# Autodesk Inventor assembly: 飛び出す奴
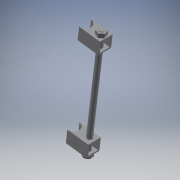
[picture p0: Inventor's stored thumbnail of the model, 180x180]
Saved by Autodesk Inventor 2018 (Build 220112000, 112)
## iProperties
Created: 2017-09-10
Part Number: 飛び出す奴
Material: 一般
Document SubType Name: Assembly
Designer: Kenta
Author: Kenta
## Documents named in this file (4)
- C:\Users\Kenta\Documents\workspace\rbbr\cart\シャーシ\飛び出す奴上.iam
- C:\Users\Kenta\Documents\workspace\rbbr\cart\シャーシ\左右に飛び出すパイプ.ipt
- C:\Users\Kenta\Documents\workspace\rbbr\cart\シャーシ\14mmパイプ.ipt
- C:\Users\Kenta\Documents\workspace\rbbr\cart\シャーシ\hn1_12.ipt
## Components (5 placed, 3 different names)
1. 左右に飛び出すパイプ:1 — フラッシュ:3, メイト:7
2. 14mmパイプ:1 — メイト:3, メイト:6, フラッシュ:4, フラッシュ:5
3. 左右に飛び出すパイプ:2 — フラッシュ:3, メイト:5
4. hn1_12:1 — メイト:3, メイト:5, フラッシュ:5
5. hn1_12:2 — メイト:6, メイト:7, フラッシュ:4
## Relationships (9: Mate 6, Flush 3)
- [Mate]: 左右に飛び出すパイプ:1 ↔ 14mmパイプ:1
- [Mate]: 14mmパイプ:1 ↔ 左右に飛び出すパイプ:2
- フラッシュ:3 [Flush]: 左右に飛び出すパイプ:1 ↔ 左右に飛び出すパイプ:2
- メイト:3 [Mate]: 14mmパイプ:1 ↔ hn1_12:1
- メイト:5 [Mate]: 左右に飛び出すパイプ:2 ↔ hn1_12:1
- メイト:6 [Mate]: 14mmパイプ:1 ↔ hn1_12:2
- メイト:7 [Mate]: 左右に飛び出すパイプ:1 ↔ hn1_12:2
- フラッシュ:4 [Flush] (1 mm): 14mmパイプ:1 ↔ hn1_12:2
- フラッシュ:5 [Flush] (-1 mm): 14mmパイプ:1 ↔ hn1_12:1
